# Autodesk Inventor assembly: UNLHEP-14-A-01-005_HdiGlueWeight
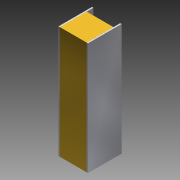
[picture p0: Inventor's stored thumbnail of the model, 180x180]
Saved by Autodesk Inventor 2013 (Build 170138000, 138)
## iProperties
Created: 2014-01-06
Part Number: UNLHEP-14-A-01-005_HdiGlueWeight
Document SubType Name: Assembly
Designer: Frank Meier
Project: UNL Pixel Phase I
Author: Frank Meier
## Documents named in this file (3)
- C:\Users\Frank Meier\Documents\Inventor\Delvotec-Saugplatte\UNLHEP-14-01-A-005_HdiGlueWeight.iam
- C:\Users\Frank Meier\Documents\Inventor\Delvotec-Saugplatte\UNLHEP-14-01-P-009_BrassWeight.ipt
- C:\Users\Frank Meier\Documents\Inventor\Delvotec-Saugplatte\UNLHEP-14-01-P-010_WeightBlade.ipt
## Components (3 placed, 2 different names)
1. MS-Gewicht:1 — Passend:1, Fluchtend:1, Fluchtend:2, Passend:2, Fluchtend:3, Fluchtend:4
2. Niederdrücker:1 — Passend:1, Fluchtend:1, Fluchtend:2
3. Niederdrücker:2 — Passend:2, Fluchtend:3, Fluchtend:4
## Relationships (6: Flush 4, Mate 2)
- Passend:1 [Mate]: MS-Gewicht:1 ↔ Niederdrücker:1
- Fluchtend:1 [Flush]: MS-Gewicht:1 ↔ Niederdrücker:1
- Fluchtend:2 [Flush]: MS-Gewicht:1 ↔ Niederdrücker:1
- Passend:2 [Mate]: MS-Gewicht:1 ↔ Niederdrücker:2
- Fluchtend:3 [Flush]: MS-Gewicht:1 ↔ Niederdrücker:2
- Fluchtend:4 [Flush]: MS-Gewicht:1 ↔ Niederdrücker:2
